# Autodesk Inventor assembly: EndPhalangeAssembly
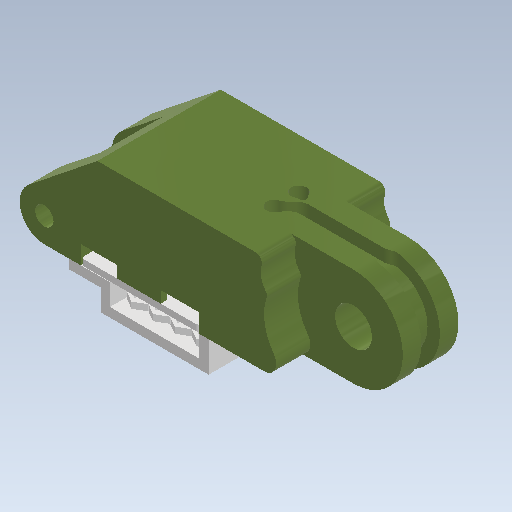
[picture p0: Inventor's stored thumbnail of the model, 512x512]
Saved by Autodesk Inventor 2020 (Build 240168000, 168)
## iProperties
Created: 2019-10-19
Part Number: EndPhalangeAssembly
Document SubType Name: Assembly
Designer: ayad493
Author: ayad493
## Documents named in this file (4)
- C:\Users\Ajay Yadiki\Desktop\Project Gripper\EndPhalangeAssembly.iam
- C:\Users\Ajay Yadiki\Desktop\Project Gripper\EndFlange.ipt
- C:\Users\Ajay Yadiki\Desktop\Project Gripper\EndPhalangeGrip.ipt
- C:\Users\Ajay Yadiki\Desktop\Project Gripper\EndPhalange_grip_support.ipt
## Components (3 placed, 3 different names)
1. EndFlange:1 — Mate:1, Flush:1, Mate:2, Mate:3, Flush:2, Flush:3
2. EndPhalangeGrip:1 — Mate:3, Flush:2, Flush:3
3. EndPhalange_grip_support:1 — Mate:1, Flush:1, Mate:2
## Relationships (6: Mate 3, Flush 3)
- Mate:1: EndFlange:1 ↔ EndPhalange_grip_support:1
- Flush:1: EndFlange:1 ↔ EndPhalange_grip_support:1
- Mate:2 (0.1 mm): EndFlange:1 ↔ EndPhalange_grip_support:1
- Mate:3: EndFlange:1 ↔ EndPhalangeGrip:1
- Flush:2: EndFlange:1 ↔ EndPhalangeGrip:1
- Flush:3: EndFlange:1 ↔ EndPhalangeGrip:1
